# Autodesk Inventor assembly: X-Axis Assembly Machine
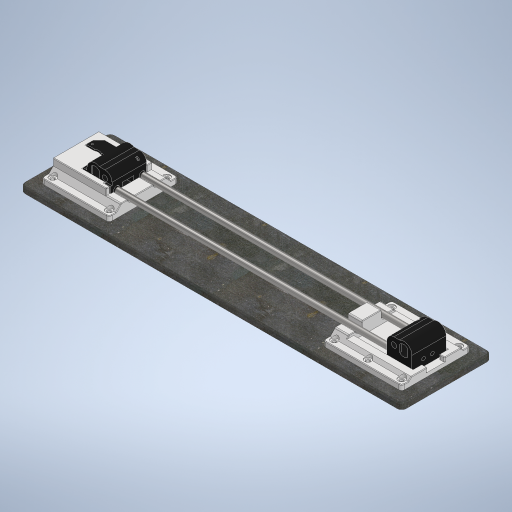
[picture p0: Inventor's stored thumbnail of the model, 512x512]
Saved by Autodesk Inventor 2023 (Build 270158000, 158)
## iProperties
Created: 2023-07-27
Part Number: X-Axis Assembly Machine
Document SubType Name: Assembly
Designer: Parker
Author: Parker
## Documents named in this file (10)
- D:\000 - PEPCORP CLOUD\00- Legacy\Designs\MK3PRO P1\Assembly Systems\X-Axis Assembly Machine.iam
- D:\000 - PEPCORP CLOUD\00- Legacy\Designs\MK3PRO P1\X-Axis\X-AXIS ASSEMBLY.iam
- D:\000 - PEPCORP CLOUD\00- Legacy\Designs\MK3PRO P1\X-Axis\X-AXIS ROD.ipt
- D:\000 - PEPCORP CLOUD\00- Legacy\Designs\MK3PRO P1\X-Axis\X-End-motor v0.3.ipt
- X-End-motor v0.4.ipt
- D:\000 - PEPCORP CLOUD\00- Legacy\Designs\MK3PRO P1\X-Axis\X-End-Idler v0.3.ipt
- X-End-Idler v0.4.ipt
- D:\000 - PEPCORP CLOUD\00- Legacy\Designs\MK3PRO P1\Assembly Systems\X-Axis Assembly Machine\X-Idler Jig v0.1.ipt
- D:\000 - PEPCORP CLOUD\00- Legacy\Designs\MK3PRO P1\Assembly Systems\X-Axis Assembly Machine\X-Motor Jig v0.1.ipt
- D:\000 - PEPCORP CLOUD\00- Legacy\Designs\MK3PRO P1\Assembly Systems\X-Axis Assembly Machine\MountingPlate.ipt
## Components (8 placed, 7 different names)
1. Finished Product [sub-assembly]
2. X-AXIS ROD:1
3. X-AXIS ROD:2
4. X-End-motor v0.4:1
5. X-End-Idler v0.4:1
6. X-Idler Jig v0.1:1 — Flush:2, Flush:3
7. X-Motor Jig v0.1:1 — Flush:4
8. MountingPlate:1 — Flush:5
## Relationships (5: Flush 5)
- Flush:1 (-10 mm)
- Flush:2: X-Idler Jig v0.1:1
- Flush:3: X-Idler Jig v0.1:1
- Flush:4: X-Motor Jig v0.1:1
- Flush:5: MountingPlate:1
